# Autodesk Inventor assembly: Futterschüssel_Platte
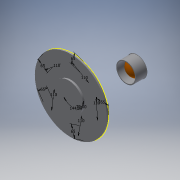
[picture p0: Inventor's stored thumbnail of the model, 180x180]
Saved by Autodesk Inventor 2016 (Build 200138000, 138)
## iProperties
Created: 2017-09-29
Part Number: Futterschüssel_Platte
Material: Generisch
Document SubType Name: Assembly
Designer: Dominik
Author: Dominik
## Documents named in this file (4)
- C:\Users\Dominik\Desktop\Diplomarbeit\Inverntorskizzen\Futterschüssel_Platte.iam
- C:\Users\Dominik\Desktop\Schule 2016-17\KÜ\2KÜ-Projekt PH\Drehplatte_Rahmenvorrrichtung.ipt
- C:\Users\Dominik\Desktop\Schule 2016-17\KÜ\2KÜ-Projekt PH\Futterschüssel_außen.ipt
- C:\Users\Dominik\Desktop\Schule 2016-17\KÜ\2KÜ-Projekt PH\Futterschüssel_innen.ipt
## Components (3 placed, 3 different names)
1. Drehplatte_Rahmenvorrrichtung:1
2. Futterschüssel_außen:1 — Passend:1, Passend:2
3. Futterschüssel_innen:1 — Passend:1, Passend:2
## Relationships (2: Mate 2)
- Passend:1 [Mate]: Futterschüssel_außen:1 ↔ Futterschüssel_innen:1
- Passend:2 [Mate]: Futterschüssel_außen:1 ↔ Futterschüssel_innen:1
